# Autodesk Inventor assembly: N20Module_MIR
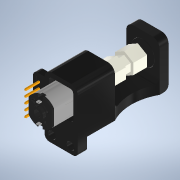
[picture p0: Inventor's stored thumbnail of the model, 180x180]
Saved by Autodesk Inventor 2022 (Build 260153000, 153)
## iProperties
Created: 2021-12-07
Part Number: N20Module_MIR
Document SubType Name: Assembly
Designer: JK
Author: JK
## Documents named in this file (6)
- C:\Users\JK\Documents\Inventor\N20 Leg Actuator\N20-Leg-Actuator\CADfiles\N20Module\N20Module_MIR.iam
- C:\Users\JK\Documents\Inventor\N20 Leg Actuator\N20-Leg-Actuator\CADfiles\N20Module\Case_MIR.ipt
- C:\Users\JK\Documents\Inventor\N20 Leg Actuator\N20-Leg-Actuator\CADfiles\N20Module\Brushed DC Motor v8_MIR.iam
- C:\Users\JK\Documents\Inventor\N20 Leg Actuator\N20-Leg-Actuator\CADfiles\N20Module\ServoPot_MIR.ipt
- C:\Users\JK\Documents\Inventor\N20 Leg Actuator\N20-Leg-Actuator\CADfiles\N20Module\Couple_MIR.ipt
- C:\Users\JK\Documents\Inventor\N20 Leg Actuator\N20-Leg-Actuator\CADfiles\N20Module\5pinheader_MIR.ipt
## Components (5 placed, 5 different names)
1. Case_MIR:1 — Coincidencia:2, Ángulo:1, Coincidencia:1, Nivelación:1, Coincidencia:7, Coincidencia:6
2. Brushed DC Motor v8_MIR:1 [sub-assembly] — Coincidencia:2, Ángulo:1, Coincidencia:1, Coincidencia:3, Coincidencia:5
3. ServoPot_MIR:1 — Coincidencia:3, Coincidencia:8
4. Couple_MIR:1 — Coincidencia:8, Coincidencia:5
5. 5pinheader_MIR:1 — Nivelación:1, Coincidencia:7, Coincidencia:6
## Relationships (9: Mate 7, Angle 1, Flush 1)
- Coincidencia:2 [Mate]: Case_MIR:1 ↔ Brushed DC Motor v8_MIR:1
- Ángulo:1 [Angle] (0 deg): Case_MIR:1 ↔ Brushed DC Motor v8_MIR:1
- Coincidencia:1 [Mate]: Case_MIR:1 ↔ Brushed DC Motor v8_MIR:1
- Coincidencia:3 [Mate]: Brushed DC Motor v8_MIR:1 ↔ ServoPot_MIR:1
- Coincidencia:8 [Mate]: ServoPot_MIR:1 ↔ Couple_MIR:1
- Coincidencia:5 [Mate]: Brushed DC Motor v8_MIR:1 ↔ Couple_MIR:1
- Nivelación:1 [Flush]: Case_MIR:1 ↔ 5pinheader_MIR:1
- Coincidencia:7 [Mate] (0.1 mm): Case_MIR:1 ↔ 5pinheader_MIR:1
- Coincidencia:6 [Mate] (0.1 mm): Case_MIR:1 ↔ 5pinheader_MIR:1
